# Autodesk Inventor assembly: Isdt
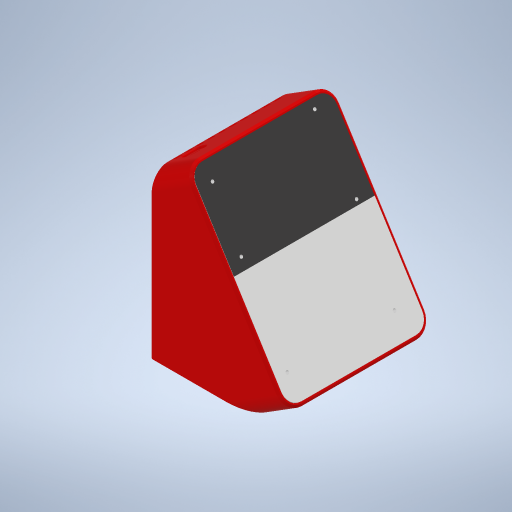
[picture p0: Inventor's stored thumbnail of the model, 512x512]
Saved by Autodesk Inventor 2023.1 (Build 271208000, 208)
## iProperties
Created: 2022-09-09
Part Number: Isdt
Document SubType Name: Assembly
Designer: Rama
Author: Rama
## Documents named in this file (7)
- C:\Users\Rama\Desktop\GitHub\Voron-2-Mods\Misc\ISDT C4 EVO\CAD\Isdt.iam
- C:\Users\Rama\Desktop\GitHub\Voron-2-Mods\Misc\ISDT C4 EVO\CAD\SRC\Isdt_Dummy.ipt
- C:\Users\Rama\Desktop\GitHub\Voron-2-Mods\Misc\ISDT C4 EVO\CAD\SRC\Housing.ipt
- C:\Users\Rama\Desktop\GitHub\Voron-2-Mods\Misc\ISDT C4 EVO\CAD\SRC\FanCover.ipt
- C:\Users\Rama\Desktop\GitHub\Voron-2-Mods\Arducam_IMX477_CM4\CM4\CAD\Source\Noctua A4x10\Noctua-Fan-NF-A4x10_40mm.iam
- C:\Users\Rama\Desktop\GitHub\Voron-2-Mods\Misc\ISDT C4 EVO\CAD\Feets.ipt
- C:\Users\Rama\Desktop\GitHub\TrashInventor\DIN EN ISO 7050 - ST4,8 x 13 - F - H.ipt
## Components (12 placed, 6 different names)
1. Isdt_Dummy:1 — Passend:5, Passend:6, Fluchtend:4
2. Housing:1 — Fluchtend:2, Passend:1, Passend:2, Fluchtend:3, Passend:3, Passend:4, Passend:5, Passend:6, Fluchtend:4, Passend:10, Passend:11, Passend:12, Passend:13, Passend:14, Fluchtend:11
3. FanCover:1 — Fluchtend:2, Passend:1, Passend:2, Passend:7, Passend:8, Passend:9, Passend:16, Passend:17, Passend:18
4. Noctua-Fan-NF-A4x10_40mm:1 [sub-assembly] — Passend:7, Passend:8, Passend:9, Passend:15
5. Feets:1 — Fluchtend:5, Fluchtend:6, Passend:13
6. Feets:2 — Fluchtend:5, Passend:10, Passend:11
7. Feets:3 — Fluchtend:6, Fluchtend:7, Passend:14
8. Feets:4 — Fluchtend:7, Passend:12
9. DIN EN ISO 7050 - F-H ST4,8 x 13 - F - H:1 — Passend:15, Fluchtend:8, Fluchtend:9
10. DIN EN ISO 7050 - F-H ST4,8 x 13 - F - H:2 — Passend:16, Fluchtend:10
11. DIN EN ISO 7050 - F-H ST4,8 x 13 - F - H:3 — Passend:18, Fluchtend:8, Fluchtend:11
12. DIN EN ISO 7050 - F-H ST4,8 x 13 - F - H:4 — Passend:17, Fluchtend:9, Fluchtend:10
## Relationships (28: Mate 18, Flush 10)
- Fluchtend:2 [Flush]: Housing:1 ↔ FanCover:1
- Passend:1 [Mate]: Housing:1 ↔ FanCover:1
- Passend:2 [Mate]: Housing:1 ↔ FanCover:1
- Fluchtend:3 [Flush]: Housing:1
- Passend:3 [Mate]: Housing:1
- Passend:4 [Mate]: Housing:1
- Passend:5 [Mate]: Isdt_Dummy:1 ↔ Housing:1
- Passend:6 [Mate]: Isdt_Dummy:1 ↔ Housing:1
- Fluchtend:4 [Flush]: Isdt_Dummy:1 ↔ Housing:1
- Passend:7 [Mate]: FanCover:1 ↔ Noctua-Fan-NF-A4x10_40mm:1
- Passend:8 [Mate]: FanCover:1 ↔ Noctua-Fan-NF-A4x10_40mm:1
- Passend:9 [Mate]: FanCover:1 ↔ Noctua-Fan-NF-A4x10_40mm:1
- Fluchtend:5 [Flush]: Feets:1 ↔ Feets:2
- Fluchtend:6 [Flush]: Feets:1 ↔ Feets:3
- Fluchtend:7 [Flush]: Feets:3 ↔ Feets:4
- Passend:10 [Mate]: Housing:1 ↔ Feets:2
- Passend:11 [Mate]: Housing:1 ↔ Feets:2
- Passend:12 [Mate]: Housing:1 ↔ Feets:4
- Passend:13 [Mate]: Housing:1 ↔ Feets:1
- Passend:14 [Mate]: Housing:1 ↔ Feets:3
- Passend:15 [Mate]: Noctua-Fan-NF-A4x10_40mm:1 ↔ DIN EN ISO 7050 - F-H ST4,8 x 13 - F - H:1
- Passend:16 [Mate]: FanCover:1 ↔ DIN EN ISO 7050 - F-H ST4,8 x 13 - F - H:2
- Passend:17 [Mate]: FanCover:1 ↔ DIN EN ISO 7050 - F-H ST4,8 x 13 - F - H:4
- Passend:18 [Mate]: FanCover:1 ↔ DIN EN ISO 7050 - F-H ST4,8 x 13 - F - H:3
- Fluchtend:8 [Flush]: DIN EN ISO 7050 - F-H ST4,8 x 13 - F - H:1 ↔ DIN EN ISO 7050 - F-H ST4,8 x 13 - F - H:3
- Fluchtend:9 [Flush]: DIN EN ISO 7050 - F-H ST4,8 x 13 - F - H:1 ↔ DIN EN ISO 7050 - F-H ST4,8 x 13 - F - H:4
- Fluchtend:10 [Flush]: DIN EN ISO 7050 - F-H ST4,8 x 13 - F - H:2 ↔ DIN EN ISO 7050 - F-H ST4,8 x 13 - F - H:4
- Fluchtend:11 [Flush] (-0.5 mm): Housing:1 ↔ DIN EN ISO 7050 - F-H ST4,8 x 13 - F - H:3
